# Autodesk Inventor assembly: Gel tray
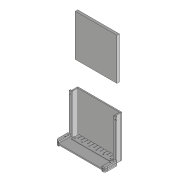
[picture p0: Inventor's stored thumbnail of the model, 180x180]
Saved by Autodesk Inventor 2020 (Build 240168000, 168)
## iProperties
Created: 2022-04-26
Part Number: Gel tray
Document SubType Name: Assembly
Designer: ferrerx
Author: ferrerx
## Documents named in this file (9)
- C:\Users\ferrerx\Desktop\Projects\Boulton Lab\Gel tray.iam
- C:\Users\ferrerx\Desktop\Projects\Boulton Lab\Gel base.ipt
- C:\Users\ferrerx\Desktop\Projects\Boulton Lab\Gel top.ipt
- C:\Users\ferrerx\Desktop\Projects\Boulton Lab\Gel wall.ipt
- C:\Users\ferrerx\Desktop\Projects\Boulton Lab\Gel.ipt
- C:\Users\ferrerx\Desktop\Projects\Boulton Lab\Comb2.ipt
- C:\Users\ferrerx\Desktop\Projects\Boulton Lab\Comb.ipt
- C:\Users\ferrerx\Desktop\Projects\Boulton Lab\Comb3.ipt
- C:\Users\ferrerx\Desktop\Projects\Boulton Lab\Comb4.ipt
## Components (14 placed, 8 different names)
1. Gel base:1 — Mate:1, Flush:1, Flush:2, Mate:3, Flush:5, Flush:6, Mate:5
2. Gel top:1 — Mate:4, Flush:7, Flush:8, Mate:28, Mate:29
3. Gel top:2 — Mate:2, Flush:3, Flush:4, Mate:30
4. Gel wall:1 — Mate:3, Flush:5, Flush:6, Mate:4, Flush:7, Flush:8, Mate:6
5. Gel wall:2 — Mate:1, Flush:1, Flush:2, Mate:2, Flush:3, Flush:4
6. Gel:1 — Mate:5, Mate:6
7. Comb2:1 — Mate:7, Mate:8, Mate:9, Mate:10, Mate:11, Mate:12, Mate:13, Mate:14, Mate:15, Mate:16, Mate:17, Mate:18, Mate:19, Mate:20, Mate:21, Mate:22, Mate:24, Mate:25, Mate:26, Mate:28
8. Comb:1 — Mate:7, Mate:8, Mate:9
9. Comb3:1 — Mate:12, Mate:13, Mate:14
10. Comb3:2 — Mate:10, Mate:11, Mate:15
11. Comb3:3 — Mate:16, Mate:17, Mate:27
12. Comb3:4 — Mate:18, Mate:19, Mate:23
13. Comb4:1 — Mate:20, Mate:21, Mate:22, Mate:23, Mate:29
14. Comb4:2 — Mate:24, Mate:25, Mate:26, Mate:27, Mate:30
## Relationships (38: Mate 30, Flush 8)
- Mate:1: Gel base:1 ↔ Gel wall:2
- Flush:1: Gel base:1 ↔ Gel wall:2
- Flush:2: Gel base:1 ↔ Gel wall:2
- Mate:2: Gel top:2 ↔ Gel wall:2
- Flush:3: Gel top:2 ↔ Gel wall:2
- Flush:4: Gel top:2 ↔ Gel wall:2
- Mate:3: Gel base:1 ↔ Gel wall:1
- Flush:5: Gel base:1 ↔ Gel wall:1
- Flush:6: Gel base:1 ↔ Gel wall:1
- Mate:4: Gel top:1 ↔ Gel wall:1
- Flush:7: Gel top:1 ↔ Gel wall:1
- Flush:8: Gel top:1 ↔ Gel wall:1
- Mate:5: Gel base:1 ↔ Gel:1
- Mate:6: Gel wall:1 ↔ Gel:1
- Mate:7: Comb2:1 ↔ Comb:1
- Mate:8: Comb2:1 ↔ Comb:1
- Mate:9: Comb2:1 ↔ Comb:1
- Mate:10: Comb2:1 ↔ Comb3:2
- Mate:11: Comb2:1 ↔ Comb3:2
- Mate:12: Comb2:1 ↔ Comb3:1
- Mate:13: Comb2:1 ↔ Comb3:1
- Mate:14: Comb2:1 ↔ Comb3:1
- Mate:15: Comb2:1 ↔ Comb3:2
- Mate:16: Comb2:1 ↔ Comb3:3
- Mate:17: Comb2:1 ↔ Comb3:3
- Mate:18: Comb2:1 ↔ Comb3:4
- Mate:19: Comb2:1 ↔ Comb3:4
- Mate:20: Comb2:1 ↔ Comb4:1
- Mate:21: Comb2:1 ↔ Comb4:1
- Mate:22: Comb2:1 ↔ Comb4:1
- Mate:23: Comb3:4 ↔ Comb4:1
- Mate:24: Comb2:1 ↔ Comb4:2
- Mate:25: Comb2:1 ↔ Comb4:2
- Mate:26: Comb2:1 ↔ Comb4:2
- Mate:27: Comb3:3 ↔ Comb4:2
- Mate:28: Gel top:1 ↔ Comb2:1
- Mate:29: Gel top:1 ↔ Comb4:1
- Mate:30: Gel top:2 ↔ Comb4:2
